# Autodesk Inventor assembly: Ensamble bomba
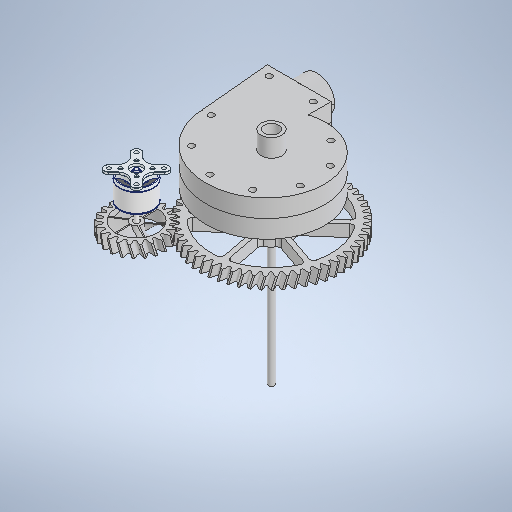
[picture p0: Inventor's stored thumbnail of the model, 512x512]
Saved by Autodesk Inventor 2025.3 (Build 293356000, 356)
## iProperties
Created: 2025-11-12
Part Number: Ensamble bomba
Document SubType Name: Assembly
Designer: juanm
Author: juanm
## Documents named in this file (8)
- C:\Users\juanm\Documents\Inventor\Turbo\Ensamble bomba.iam
- C:\Users\juanm\Documents\Inventor\Turbo\Rodete_4000RPM_2LS.ipt
- C:\Users\juanm\Documents\Inventor\Turbo\Base voluta.ipt
- C:\Users\juanm\Documents\Inventor\Turbo\Tapa voluta.ipt
- C:\Users\juanm\Documents\Inventor\Turbo\Eje 5mm.ipt
- C:\Users\juanm\Documents\Inventor\Turbo\Engrane.ipt
- C:\Users\juanm\Documents\Inventor\Turbo\Motor con soporte\Motor con soporte\Motor con soporte.iam
- C:\Users\juanm\Documents\Inventor\Turbo\Pinon.ipt
## Components (7 placed, 7 different names)
1. Rodete_4000RPM_2LS:1 — Insert:1
2. Base voluta:1 — Insert:1, Flush:1, Mate:1, Flush:2, Insert:2
3. Tapa voluta:1 — Flush:1, Mate:1, Flush:2
4. Eje 5mm:1 — Insert:2, Insert:3, Mate:2
5. Engrane:1 — Insert:3
6. Pinon:1 — Insert:4
7. Motor con soporte:1 [sub-assembly] — Mate:2, Insert:4
## Relationships (8: Insert 4, Flush 2, Mate 2)
- Insert:1 (0.5 mm): Rodete_4000RPM_2LS:1 ↔ Base voluta:1
- Flush:1: Base voluta:1 ↔ Tapa voluta:1
- Mate:1: Base voluta:1 ↔ Tapa voluta:1
- Flush:2: Base voluta:1 ↔ Tapa voluta:1
- Insert:2 (-30 mm): Base voluta:1 ↔ Eje 5mm:1
- Insert:3 (110 mm): Eje 5mm:1 ↔ Engrane:1
- Mate:2 (80 mm): Eje 5mm:1 ↔ Motor con soporte:1
- Insert:4 (9 mm): Pinon:1 ↔ Motor con soporte:1
